# Autodesk Inventor assembly: Assembly9
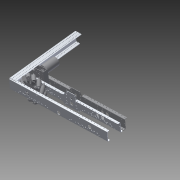
[picture p0: Inventor's stored thumbnail of the model, 180x180]
Saved by Autodesk Inventor 2015 (Build 190159000, 159)
## iProperties
Created: 2016-01-12
Part Number: Assembly9
Document SubType Name: Assembly
Designer: Applegate
Author: Applegate
## Documents named in this file (5)
- C:\Users\Applegate\Desktop\Chassy_Wheeled\Assembly\Assembly9.iam
- C:\Users\Applegate\Downloads\Imported Components\AM14U3+Long+REV1-1\AM14U3 Inside Sheet Rev2.ipt
- C:\Users\Applegate\Desktop\Chassy_Wheeled\Assembly\GearBox and Mec.iam
- C:\Users\Applegate\Downloads\Imported Components\AM14U3+Long+REV1-1\AM14U3 Outside Sheet Rev1_DefaultSM-FLAT-PATTERN.ipt
- C:\Users\Applegate\Downloads\Imported Components\AM14U3+Long+REV1-1\AM14U3 End Sheet Long.ipt
## Components (5 placed, 4 different names)
1. AM14U3 Inside Sheet Rev2:1 — Rotational:1, Flush:1
2. GearBox and Mec:1 [sub-assembly] — Rotational:1, Rotational:2, Cylindrical:1
3. AM14U3 Inside Sheet Rev2:2 — Rotational:2, Flush:1, Flush:2, Rotational:5
4. AM14U3 Outside Sheet Rev1_DefaultSM-FLAT-PATTERN:1 — Cylindrical:1, Flush:2, Rotational:3, Rotational:4
5. AM14U3 End Sheet Long:1 — Rotational:3, Rotational:4, Rotational:5
## Relationships (8: RevoluteJoint 5, Flush 2, CylindricalJoint 1)
- Rotational:1 [RevoluteJoint]: AM14U3 Inside Sheet Rev2:1 ↔ GearBox and Mec:1
- Rotational:2 [RevoluteJoint]: GearBox and Mec:1 ↔ AM14U3 Inside Sheet Rev2:2
- Flush:1: AM14U3 Inside Sheet Rev2:1 ↔ AM14U3 Inside Sheet Rev2:2
- Cylindrical:1: GearBox and Mec:1 ↔ AM14U3 Outside Sheet Rev1_DefaultSM-FLAT-PATTERN:1
- Flush:2: AM14U3 Inside Sheet Rev2:2 ↔ AM14U3 Outside Sheet Rev1_DefaultSM-FLAT-PATTERN:1
- Rotational:3 [RevoluteJoint]: AM14U3 Outside Sheet Rev1_DefaultSM-FLAT-PATTERN:1 ↔ AM14U3 End Sheet Long:1
- Rotational:4 [RevoluteJoint]: AM14U3 Outside Sheet Rev1_DefaultSM-FLAT-PATTERN:1 ↔ AM14U3 End Sheet Long:1
- Rotational:5 [RevoluteJoint]: AM14U3 Inside Sheet Rev2:2 ↔ AM14U3 End Sheet Long:1
